# Autodesk Inventor assembly: RoueV3
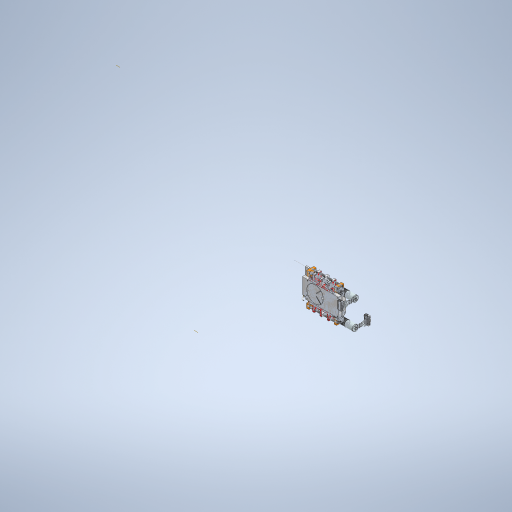
[picture p0: Inventor's stored thumbnail of the model, 512x512]
Saved by Autodesk Inventor 2023 (Build 270158000, 158)
## iProperties
Created: 2023-04-29
Part Number: RoueV3
Document SubType Name: Assembly
Designer: Nathann
Author: Nathann
## Documents named in this file (11)
- C:\Users\Nathann\ClawdDrive\Objet3D\IminaProbe\V3Roue\RoueV3.iam
- C:\Users\Nathann\ClawdDrive\Objet3D\IminaProbe\V3Roue\CapacitiveSensor.ipt
- C:\Users\Nathann\ClawdDrive\Objet3D\IminaProbe\V3Roue\RoueV3partA.ipt
- C:\Users\Nathann\ClawdDrive\Objet3D\IminaProbe\V3Roue\RoueV3PartB.ipt
- C:\Users\Nathann\ClawdDrive\Objet3D\IminaProbe\V3Roue\RoueV3PartC.ipt
- C:\Users\Nathann\ClawdDrive\Objet3D\IminaProbe\V3Roue\Probe.ipt
- C:\Users\Nathann\ClawdDrive\Objet3D\IminaProbe\V3Roue\91292A832_18-8 Stainless Steel Socket Head Screw.ipt
- C:\Users\Nathann\ClawdDrive\Objet3D\3DPrinter\inventor\AngleScrewBlocActuator.ipt
- C:\Users\Nathann\Documents\Inventor\Content Center Files\R2023\en-US\AS 1420\AS 1420 - 1973 - M3 x 16.ipt
- C:\Users\Nathann\ClawdDrive\Objet3D\3DPrinter\inventor\Sprint.ipt
- C:\Users\Nathann\ClawdDrive\Objet3D\IminaProbe\LinearAxis\DifferentialLinearActuator.ipt
## Components (20 placed, 10 different names)
1. CapacitiveSensor:1 — Flush:11, Mate:3, Insert:3, Insert:4
2. RoueV3partA:1 — Flush:1, Flush:11, Mate:3, Insert:1
3. RoueV3PartB:1 — Flush:1, Flush:2, Insert:1, Insert:2, Flush:12, Insert:13, Insert:14
4. RoueV3PartC:1 — Flush:2, Insert:2, Insert:6, Insert:7, Insert:8, Insert:9, Insert:10, Insert:11, Insert:12
5. Probe:1
6. DifferentialLinearActuator:13
7. DifferentialLinearActuator:14
8. 91292A832_18-8 Stainless Steel Socket Head Screw:1 — Insert:3
9. 91292A832_18-8 Stainless Steel Socket Head Screw:2 — Insert:4
10. AngleScrewBlocActuator:1 — Flush:12
11. 91292A832_18-8 Stainless Steel Socket Head Screw:3 — Insert:6
12. 91292A832_18-8 Stainless Steel Socket Head Screw:4 — Insert:7
13. AS 1420 - Metric M3 x 16:1 — Insert:8
14. AS 1420 - Metric M3 x 16:2 — Insert:9
15. AS 1420 - Metric M3 x 16:3 — Insert:10
16. AS 1420 - Metric M3 x 16:4 — Insert:11
17. AS 1420 - Metric M3 x 16:5 — Insert:12
18. 91292A832_18-8 Stainless Steel Socket Head Screw:5 — Insert:14
19. 91292A832_18-8 Stainless Steel Socket Head Screw:6 — Insert:13
20. Sprint:1
## Relationships (29: Insert 16, Flush 10, Mate 3)
- Flush:1: RoueV3partA:1 ↔ RoueV3PartB:1
- Flush:2: RoueV3PartB:1 ↔ RoueV3PartC:1
- [Mate]: RoueV3partA:1 ↔ DifferentialLinearActuator:13
- [Flush]: RoueV3partA:1 ↔ DifferentialLinearActuator:13
- [Mate]: RoueV3partA:1 ↔ DifferentialLinearActuator:14
- [Flush]: RoueV3partA:1 ↔ DifferentialLinearActuator:14
- [Flush] (10 mm): RoueV3partA:1 ↔ DifferentialLinearActuator:14
- [Flush] (10 mm): RoueV3partA:1 ↔ DifferentialLinearActuator:13
- Flush:11: CapacitiveSensor:1 ↔ RoueV3partA:1
- Mate:3: CapacitiveSensor:1 ↔ RoueV3partA:1
- Insert:1: RoueV3partA:1 ↔ RoueV3PartB:1
- Insert:2: RoueV3PartB:1 ↔ RoueV3PartC:1
- Insert:3: CapacitiveSensor:1 ↔ 91292A832_18-8 Stainless Steel Socket Head Screw:1
- Insert:4: CapacitiveSensor:1 ↔ 91292A832_18-8 Stainless Steel Socket Head Screw:2
- Flush:12: RoueV3PartB:1 ↔ AngleScrewBlocActuator:1
- [Insert]: DifferentialLinearActuator:14 ↔ AngleScrewBlocActuator:1
- Insert:6: RoueV3PartC:1 ↔ 91292A832_18-8 Stainless Steel Socket Head Screw:3
- Insert:7: RoueV3PartC:1 ↔ 91292A832_18-8 Stainless Steel Socket Head Screw:4
- Insert:8: RoueV3PartC:1 ↔ AS 1420 - Metric M3 x 16:1
- Insert:9: RoueV3PartC:1 ↔ AS 1420 - Metric M3 x 16:2
- Insert:10: RoueV3PartC:1 ↔ AS 1420 - Metric M3 x 16:3
- Insert:11: RoueV3PartC:1 ↔ AS 1420 - Metric M3 x 16:4
- Insert:12: RoueV3PartC:1 ↔ AS 1420 - Metric M3 x 16:5
- Insert:13: RoueV3PartB:1 ↔ 91292A832_18-8 Stainless Steel Socket Head Screw:6
- Insert:14: RoueV3PartB:1 ↔ 91292A832_18-8 Stainless Steel Socket Head Screw:5
- [Insert]: RoueV3PartC:1 ↔ DifferentialLinearActuator:13
- [Insert]: RoueV3PartC:1 ↔ DifferentialLinearActuator:14
- [Flush]: RoueV3PartC:1 ↔ DifferentialLinearActuator:13
- [Flush]: RoueV3PartC:1 ↔ DifferentialLinearActuator:14
